# Autodesk Inventor assembly: GearedUpper
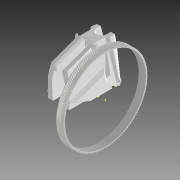
[picture p0: Inventor's stored thumbnail of the model, 180x180]
Saved by Autodesk Inventor 2020 (Build 240168000, 168)
## iProperties
Created: 2020-09-19
Part Number: GearedUpper
Document SubType Name: Assembly
Designer: DDeGo
Author: DDeGo
## Documents named in this file (3)
- C:\Users\DDeGo\Documents\Drew\Projects\Nerf Aim Assist\Cad\GearedUpper.iam
- C:\Users\DDeGo\Documents\Drew\Projects\Nerf Aim Assist\ESPER\EUpper_Alt.ipt
- C:\Users\DDeGo\Documents\Drew\Projects\Nerf Aim Assist\Cad\144 Tooth Herringbone semicircle.ipt
## Components (2 placed, 2 different names)
1. EUpper_Alt:1 — Mate:1, Mate:2
2. 144 Tooth Herringbone semicircle:1 — Mate:1, Mate:2
## Relationships (2: Mate 2)
- Mate:1: EUpper_Alt:1 ↔ 144 Tooth Herringbone semicircle:1
- Mate:2: EUpper_Alt:1 ↔ 144 Tooth Herringbone semicircle:1
